# Autodesk Inventor assembly: bike
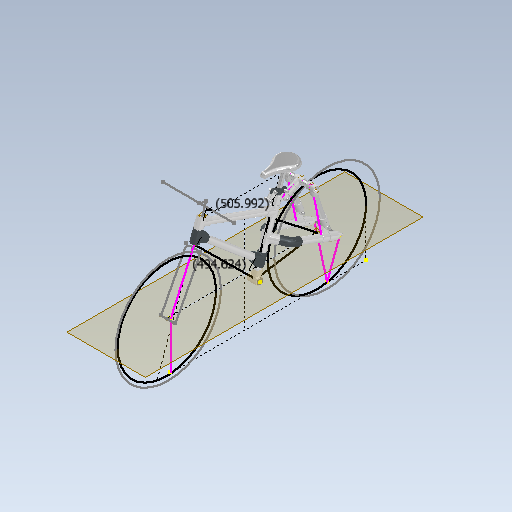
[picture p0: Inventor's stored thumbnail of the model, 512x512]
Saved by Autodesk Inventor 2021 (Build 250183000, 183)
## iProperties
RuleStatus: InUse
Created: 2020-04-29
Part Number: bike
Document SubType Name: Assembly
Designer: Hannah
Mass: 10072.6 g
Surface Area: 13426.9 cm^2
Volume: 2555.77 cm^3
Density: 3.94113 g/cm^3
BeforeDocSave0: estimate cost
Total Cost: 100
Author: Hannah
## Documents named in this file (29)
- \\Mac\Home\Documents\GitHub\AdjustaBike-2.0\CAD\bike.iam
- \\Mac\Home\Documents\GitHub\AdjustaBike-2.0\CAD\prelim bike geo.ipt
- \\Mac\Home\Documents\GitHub\AdjustaBike-2.0\CAD\bottom bracket.ipt
- \\Mac\Home\Documents\GitHub\AdjustaBike-2.0\CAD\L10-7.ipt
- \\Mac\Home\Documents\GitHub\AdjustaBike-2.0\CAD\tube-07.ipt
- \\Mac\Home\Documents\GitHub\AdjustaBike-2.0\CAD\tube-08.ipt
- \\Mac\Home\Documents\GitHub\AdjustaBike-2.0\CAD\tube-11.ipt
- \\Mac\Home\Documents\GitHub\AdjustaBike-2.0\CAD\tube-12.ipt
- \\Mac\Home\Documents\GitHub\AdjustaBike-2.0\CAD\329-7.ipt
- \\Mac\Home\Documents\GitHub\AdjustaBike-2.0\CAD\head tube.ipt
- \\Mac\Home\Documents\GitHub\AdjustaBike-2.0\CAD\LM50-7.ipt
- \\Mac\Home\Documents\GitHub\AdjustaBike-2.0\CAD\LF50-6.ipt
- \\Mac\Home\Documents\GitHub\AdjustaBike-2.0\CAD\55-7.ipt
- \\Mac\Home\Documents\GitHub\AdjustaBike-2.0\CAD\L21-7.ipt
- \\Mac\Home\Documents\GitHub\AdjustaBike-2.0\CAD\tube-13.ipt
- \\Mac\Home\Documents\GitHub\AdjustaBike-2.0\CAD\LF50-7.ipt
- \\Mac\Home\Documents\GitHub\AdjustaBike-2.0\CAD\L10-6.ipt
- \\Mac\Home\Documents\GitHub\AdjustaBike-2.0\CAD\tube-14.ipt
- \\Mac\Home\Documents\GitHub\AdjustaBike-2.0\CAD\L114-6.ipt
- \\Mac\Home\Documents\GitHub\AdjustaBike-2.0\CAD\saddle.ipt
- \\Mac\Home\Documents\GitHub\AdjustaBike-2.0\CAD\M51-5.ipt
- \\Mac\Home\Documents\GitHub\AdjustaBike-2.0\CAD\link.ipt
- \\Mac\Home\Documents\GitHub\AdjustaBike-2.0\CAD\LM51-7.ipt
- \\Mac\Home\Documents\GitHub\AdjustaBike-2.0\CAD\fasteners\DIN 1587 - M10 x 1.5.ipt
- \\Mac\Home\Documents\GitHub\AdjustaBike-2.0\CAD\fasteners\DIN EN ISO 7089 -  10.ipt
- \\Mac\Home\Documents\GitHub\AdjustaBike-2.0\CAD\fasteners\BS EN ISO 4762 - M10 x 35.ipt
- \\Mac\Home\Documents\GitHub\AdjustaBike-2.0\CAD\fasteners\BS EN ISO 4762 - M10 x 45.ipt
- \\Mac\Home\Documents\GitHub\AdjustaBike-2.0\CAD\tube-01.ipt
- \\Mac\Home\Documents\GitHub\AdjustaBike-2.0\CAD\bike sketch.ipt
## Components (69 placed, 28 different names)
1. bike sketch:1 — Flush:126, Flush:127, Flush:128, Mate:236, Mate:237, Mate:238, Mate:239, Mate:240, Mate:241, Mate:242, Mate:243, Mate:244, Mate:245, Mate:246, Mate:247, Mate:248, Mate:249, Mate:250, Mate:251, Mate:252, Mate:253, Mate:254, Mate:255, Mate:256, Mate:257, Mate:258, Mate:259, Mate:260
2. prelim bike geo:1 — Mate:1, Mate:2, Angle:1, Mate:41
3. seat tube:1 — Mate:7, Tangent:1, Flush:9, Angle:2, Mate:8, Angle:5, Mate:17, Tangent:7, Tangent:8, Mate:28, Mate:52, Flush:21, Mate:106, Mate:240
4. down tube:1 — Flush:10, Angle:3, Tangent:2, Mate:11, Tangent:3, Angle:4, Mate:12, Mate:242
5. top tube:1 — Mate:16, Tangent:4, Mate:18, Mate:241
6. seatstay:1 — Mate:91, Mate:93, Mate:97, Mate:245
7. seatstay:2 — Mate:45, Mate:47, Mate:82, Tangent:9, Mate:246
8. seatstay spacer:1 — Mate:89, Mate:90, Mate:92, Mate:100, Tangent:9, Mate:254, Mate:255
9. chainstay:2 — Mate:59, Mate:64, Angle:13, Mate:74, Mate:76, Mate:79, Mate:248
10. chainstay:1 — Mate:58, Mate:62, Angle:12, Mate:75, Mate:77, Mate:247
11. chainstay spacer:1 — Tangent:8, Mate:55, Mate:57, Mate:61, Mate:250
12. chainstay spacer:2 — Tangent:7, Mate:54, Mate:56, Mate:63, Mate:249
13. L10-7:1 — Mate:6, Flush:2, Mate:7, Mate:9
14. L10-7:2 — Mate:17, Mate:18, Mate:261
15. L10-7:3 — Mate:15, Flush:13, Flush:14, Mate:16, Mate:239, Mate:258
16. LM51-7:1 — Mate:28, Flush:16, Mate:69, Flush:20, Flush:21, Flush:22, Mate:107, Mate:110, Mate:111, Mate:112, Mate:113, Mate:114, Mate:204, Mate:261
17. LF50-6:2 — Mate:45, Mate:47, Angle:11, Mate:83, Flush:85, Mate:175
18. L21-7:1 — Mate:52, Mate:53, Mate:54, Mate:55, Mate:60
19. L10-6:3 — Mate:91, Mate:92
20. LF50-6:4 — Mate:93, Mate:95, Mate:96, Mate:97, Mate:150
21. L114-6:1 — Mate:98, Mate:99, Mate:100, Mate:244
22. LF50-6:3 — Mate:69, Flush:20, Mate:98, Mate:99, Mate:108, Mate:109, Mate:232, Mate:243
23. LF50-7:1 — Mate:76, Mate:79, Mate:85, Mate:94, Mate:235, Mate:236, Mate:259
24. LF50-7:2 — Mate:77, Mate:78, Mate:85, Mate:86, Mate:260
25. LM50-7:3 — Mate:75, Mate:83, Flush:85, Mate:86
26. LM50-7:4 — Mate:74, Mate:94, Mate:95, Mate:96
27. L10-6:1 — Mate:82, Mate:89
28. saddle and seatpost:1 — Mate:106, Flush:116
29. head tube:1 — Mate:14, Flush:11, Flush:12, Angle:5, Mate:15, Flush:13, Tangent:4, Mate:237, Mate:257, Mate:262, Mate:263
30. bottom bracket:1 — Mate:4, Flush:1, Mate:5, Mate:6, Tangent:1, Mate:251, Mate:252, Mate:256
31. link:1 — Mate:107, Mate:109, Mate:226, Mate:233
32. link:2 — Mate:111, Mate:113
33. link:3 — Mate:108, Mate:112, Mate:218, Mate:234
34. link:4 — Mate:110, Mate:114, Mate:189
35. DIN 1587 - M10 x 1.5:1 — Mate:162
36. DIN EN ISO 7089 -  10:1
37. BS EN ISO 4762 - M10 x 35:1 — Mate:150, Mate:162
38. DIN EN ISO 7089 -  10:2
39. DIN 1587 - M10 x 1.5:2 — Mate:164
40. DIN EN ISO 7089 -  10:3
41. BS EN ISO 4762 - M10 x 35:2 — Mate:164, Mate:175
42. DIN EN ISO 7089 -  10:4
43. DIN 1587 - M10 x 1.5:3 — Mate:178
44. DIN EN ISO 7089 -  10:5
45. BS EN ISO 4762 - M10 x 35:3 — Mate:178, Mate:189
46. DIN EN ISO 7089 -  10:6
47. DIN 1587 - M10 x 1.5:4 — Mate:201
48. DIN EN ISO 7089 -  10:7
49. BS EN ISO 4762 - M10 x 35:4 — Mate:201, Mate:204
50. DIN EN ISO 7089 -  10:8
51. DIN EN ISO 7089 -  10:11 — Mate:216, Mate:220
52. DIN EN ISO 7089 -  10:12 — Mate:215, Mate:219, Mate:220
53. DIN EN ISO 7089 -  10:13 — Mate:217, Mate:218, Mate:219
54. DIN EN ISO 7089 -  10:14 — Mate:221, Mate:225
55. DIN EN ISO 7089 -  10:15 — Mate:221, Mate:222, Mate:224
56. DIN EN ISO 7089 -  10:16 — Mate:222, Mate:223, Mate:226
57. DIN 1587 - M10 x 1.5:5 — Mate:207
58. DIN EN ISO 7089 -  10:9
59. BS EN ISO 4762 - M10 x 45:1 — Mate:207, Mate:212, Mate:215, Mate:216, Mate:217, Mate:223, Mate:224, Mate:225
60. DIN EN ISO 7089 -  10:10
61. DIN 1587 - M10 x 1.5:6 — Mate:227, Mate:230
62. DIN EN ISO 7089 -  10:17 — Mate:228, Mate:229, Mate:234
63. BS EN ISO 4762 - M10 x 45:2 — Mate:227, Mate:228, Mate:229, Mate:231, Mate:232
64. DIN EN ISO 7089 -  10:18 — Mate:230, Mate:231, Mate:233, Mate:253
65. 329-7:1 — Mate:8, Mate:9, Mate:10, Angle:3, Tangent:2, Mate:11, Mate:53
66. 329-7:2 — Tangent:3, Angle:4, Mate:12, Mate:13, Mate:14, Flush:11, Mate:238
67. 55-7:1 — Mate:56, Mate:59, Mate:63, Mate:64
68. 55-7:2 — Mate:57, Mate:58, Mate:61, Mate:62
69. M51-5:1 — Mate:212
## Relationships (196: Mate 163, Flush 18, Angle 8, Tangent 7)
- Mate:1: prelim bike geo:1
- Mate:2: prelim bike geo:1
- Mate:3
- Mate:4: bottom bracket:1
- Flush:1: bottom bracket:1
- Angle:1 (0 deg): prelim bike geo:1
- Mate:5: bottom bracket:1
- Mate:6: L10-7:1 ↔ bottom bracket:1
- Flush:2: L10-7:1
- Mate:7: seat tube:1 ↔ L10-7:1
- Tangent:1: seat tube:1 ↔ bottom bracket:1
- Flush:9: seat tube:1
- Angle:2 (-70 deg): seat tube:1
- Flush:10: down tube:1
- Mate:8: seat tube:1 ↔ 329-7:1
- Mate:9 (5 mm): L10-7:1 ↔ 329-7:1
- Mate:10: 329-7:1
- Angle:3 (72 deg): down tube:1 ↔ 329-7:1
- Tangent:2: down tube:1 ↔ 329-7:1
- Mate:11: down tube:1 ↔ 329-7:1
- Tangent:3: down tube:1 ↔ 329-7:2
- Angle:4 (0 deg): down tube:1 ↔ 329-7:2
- Mate:12: down tube:1 ↔ 329-7:2
- Mate:13: 329-7:2
- Mate:14: head tube:1 ↔ 329-7:2
- Flush:11: head tube:1 ↔ 329-7:2
- Flush:12: head tube:1
- Angle:5 (0 deg): seat tube:1 ↔ head tube:1
- Mate:15: L10-7:3 ↔ head tube:1
- Flush:13: L10-7:3 ↔ head tube:1
- Flush:14: L10-7:3
- Mate:16: top tube:1 ↔ L10-7:3
- Tangent:4: top tube:1 ↔ head tube:1
- Mate:17: seat tube:1 ↔ L10-7:2
- Mate:18: top tube:1 ↔ L10-7:2
- Tangent:7: seat tube:1 ↔ chainstay spacer:2
- Tangent:8: seat tube:1 ↔ chainstay spacer:1
- Mate:28: seat tube:1 ↔ LM51-7:1
- Flush:16: LM51-7:1
- Mate:41: prelim bike geo:1
- Mate:45: seatstay:2 ↔ LF50-6:2
- Mate:47: seatstay:2 ↔ LF50-6:2
- Angle:11 (0 deg): LF50-6:2
- Mate:52: seat tube:1 ↔ L21-7:1
- Mate:53 (5 mm): L21-7:1 ↔ 329-7:1
- Mate:54: chainstay spacer:2 ↔ L21-7:1
- Mate:55: chainstay spacer:1 ↔ L21-7:1
- Mate:56: chainstay spacer:2 ↔ 55-7:1
- Mate:57: chainstay spacer:1 ↔ 55-7:2
- Mate:58: chainstay:1 ↔ 55-7:2
- Mate:59: chainstay:2 ↔ 55-7:1
- Mate:60: L21-7:1
- Mate:61 (-35 mm): chainstay spacer:1 ↔ 55-7:2
- Mate:62 (-35 mm): chainstay:1 ↔ 55-7:2
- Mate:63 (-35 mm): chainstay spacer:2 ↔ 55-7:1
- Mate:64 (-35 mm): chainstay:2 ↔ 55-7:1
- Angle:12 (0 deg): chainstay:1
- Angle:13 (0 deg): chainstay:2
- Mate:69: LM51-7:1 ↔ LF50-6:3
- Flush:20: LM51-7:1 ↔ LF50-6:3
- Flush:21: seat tube:1 ↔ LM51-7:1
- Mate:74: chainstay:2 ↔ LM50-7:4
- Mate:75: chainstay:1 ↔ LM50-7:3
- Mate:76: chainstay:2 ↔ LF50-7:1
- Mate:77: chainstay:1 ↔ LF50-7:2
- Mate:78: LF50-7:2
- Mate:79: chainstay:2 ↔ LF50-7:1
- Flush:22: LM51-7:1
- Mate:82: seatstay:2 ↔ L10-6:1
- Mate:83: LF50-6:2 ↔ LM50-7:3
- Flush:85: LF50-6:2 ↔ LM50-7:3
- Mate:85: LF50-7:1 ↔ LF50-7:2
- Mate:86 (5 mm): LF50-7:2 ↔ LM50-7:3
- Mate:89: seatstay spacer:1 ↔ L10-6:1
- Mate:90: seatstay spacer:1
- Mate:91: seatstay:1 ↔ L10-6:3
- Mate:92: seatstay spacer:1 ↔ L10-6:3
- Mate:93: seatstay:1 ↔ LF50-6:4
- Mate:94 (5 mm): LF50-7:1 ↔ LM50-7:4
- Mate:95: LF50-6:4 ↔ LM50-7:4
- Mate:96: LF50-6:4 ↔ LM50-7:4
- Mate:97: seatstay:1 ↔ LF50-6:4
- Mate:98: L114-6:1 ↔ LF50-6:3
- Mate:99: L114-6:1 ↔ LF50-6:3
- Mate:100: seatstay spacer:1 ↔ L114-6:1
- Tangent:9: seatstay:2 ↔ seatstay spacer:1
- [Mate]: saddle and seatpost:1 ↔ M51-5:1
- [Mate]: link:3 ↔ M51-5:1
- [Mate]: link:4 ↔ M51-5:1
- [Mate]: link:2 ↔ M51-5:1
- [Mate]: link:1 ↔ M51-5:1
- Mate:106: seat tube:1 ↔ saddle and seatpost:1
- Mate:107: LM51-7:1 ↔ link:1
- Mate:108: LF50-6:3 ↔ link:3
- Mate:109: LF50-6:3 ↔ link:1
- Mate:110: LM51-7:1 ↔ link:4
- Mate:111: LM51-7:1 ↔ link:2
- Mate:112: LM51-7:1 ↔ link:3
- Mate:113: LM51-7:1 ↔ link:2
- Mate:114: LM51-7:1 ↔ link:4
- Flush:116: saddle and seatpost:1
- Mate:150: LF50-6:4 ↔ BS EN ISO 4762 - M10 x 35:1
- [Mate]: DIN EN ISO 7089 -  10:1 ↔ BS EN ISO 4762 - M10 x 35:1
- [Mate]: DIN EN ISO 7089 -  10:1 ↔ BS EN ISO 4762 - M10 x 35:1
- [Mate]: LF50-6:4 ↔ DIN EN ISO 7089 -  10:1
- [Mate]: BS EN ISO 4762 - M10 x 35:1 ↔ DIN EN ISO 7089 -  10:2
- [Mate]: LF50-6:4 ↔ DIN EN ISO 7089 -  10:2
- Mate:162: DIN 1587 - M10 x 1.5:1 ↔ BS EN ISO 4762 - M10 x 35:1
- Mate:164: DIN 1587 - M10 x 1.5:2 ↔ BS EN ISO 4762 - M10 x 35:2
- [Mate]: DIN EN ISO 7089 -  10:3 ↔ BS EN ISO 4762 - M10 x 35:2
- [Mate]: DIN EN ISO 7089 -  10:3 ↔ BS EN ISO 4762 - M10 x 35:2
- [Mate]: BS EN ISO 4762 - M10 x 35:2 ↔ DIN EN ISO 7089 -  10:4
- Mate:175: LF50-6:2 ↔ BS EN ISO 4762 - M10 x 35:2
- [Mate]: LF50-6:2 ↔ DIN EN ISO 7089 -  10:3
- [Mate]: LF50-6:2 ↔ DIN EN ISO 7089 -  10:4
- Mate:178: DIN 1587 - M10 x 1.5:3 ↔ BS EN ISO 4762 - M10 x 35:3
- [Mate]: DIN EN ISO 7089 -  10:5 ↔ BS EN ISO 4762 - M10 x 35:3
- [Mate]: DIN EN ISO 7089 -  10:5 ↔ BS EN ISO 4762 - M10 x 35:3
- [Mate]: BS EN ISO 4762 - M10 x 35:3 ↔ DIN EN ISO 7089 -  10:6
- Mate:189: link:4 ↔ BS EN ISO 4762 - M10 x 35:3
- [Mate]: link:4 ↔ DIN EN ISO 7089 -  10:5
- [Mate]: link:2 ↔ DIN EN ISO 7089 -  10:6
- [Mate]: DIN 1587 - M10 x 1.5:1 ↔ DIN EN ISO 7089 -  10:2
- [Mate]: DIN 1587 - M10 x 1.5:2 ↔ DIN EN ISO 7089 -  10:4
- [Mate]: DIN 1587 - M10 x 1.5:3 ↔ DIN EN ISO 7089 -  10:6
- [Mate]: DIN EN ISO 7089 -  10:7 ↔ BS EN ISO 4762 - M10 x 35:4
- [Mate]: DIN EN ISO 7089 -  10:7 ↔ BS EN ISO 4762 - M10 x 35:4
- Mate:201: DIN 1587 - M10 x 1.5:4 ↔ BS EN ISO 4762 - M10 x 35:4
- [Mate]: DIN 1587 - M10 x 1.5:4 ↔ DIN EN ISO 7089 -  10:8
- [Mate]: BS EN ISO 4762 - M10 x 35:4 ↔ DIN EN ISO 7089 -  10:8
- Mate:204: LM51-7:1 ↔ BS EN ISO 4762 - M10 x 35:4
- [Mate]: link:4 ↔ DIN EN ISO 7089 -  10:7
- [Mate]: link:2 ↔ DIN EN ISO 7089 -  10:8
- Mate:207: DIN 1587 - M10 x 1.5:5 ↔ BS EN ISO 4762 - M10 x 45:1
- [Mate]: DIN EN ISO 7089 -  10:9 ↔ BS EN ISO 4762 - M10 x 45:1
- [Mate]: DIN EN ISO 7089 -  10:9 ↔ BS EN ISO 4762 - M10 x 45:1
- [Mate]: BS EN ISO 4762 - M10 x 45:1 ↔ DIN EN ISO 7089 -  10:10
- [Mate]: DIN 1587 - M10 x 1.5:5 ↔ DIN EN ISO 7089 -  10:10
- Mate:212: BS EN ISO 4762 - M10 x 45:1 ↔ M51-5:1
- [Mate]: link:3 ↔ DIN EN ISO 7089 -  10:9
- [Mate]: link:1 ↔ DIN EN ISO 7089 -  10:10
- Mate:215: DIN EN ISO 7089 -  10:12 ↔ BS EN ISO 4762 - M10 x 45:1
- Mate:216: DIN EN ISO 7089 -  10:11 ↔ BS EN ISO 4762 - M10 x 45:1
- Mate:217: DIN EN ISO 7089 -  10:13 ↔ BS EN ISO 4762 - M10 x 45:1
- Mate:218: link:3 ↔ DIN EN ISO 7089 -  10:13
- Mate:219: DIN EN ISO 7089 -  10:12 ↔ DIN EN ISO 7089 -  10:13
- Mate:220: DIN EN ISO 7089 -  10:11 ↔ DIN EN ISO 7089 -  10:12
- Mate:221: DIN EN ISO 7089 -  10:14 ↔ DIN EN ISO 7089 -  10:15
- Mate:222: DIN EN ISO 7089 -  10:15 ↔ DIN EN ISO 7089 -  10:16
- Mate:223: DIN EN ISO 7089 -  10:16 ↔ BS EN ISO 4762 - M10 x 45:1
- Mate:224: DIN EN ISO 7089 -  10:15 ↔ BS EN ISO 4762 - M10 x 45:1
- Mate:225: DIN EN ISO 7089 -  10:14 ↔ BS EN ISO 4762 - M10 x 45:1
- Mate:226: link:1 ↔ DIN EN ISO 7089 -  10:16
- Mate:227: DIN 1587 - M10 x 1.5:6 ↔ BS EN ISO 4762 - M10 x 45:2
- Mate:228: DIN EN ISO 7089 -  10:17 ↔ BS EN ISO 4762 - M10 x 45:2
- Mate:229: DIN EN ISO 7089 -  10:17 ↔ BS EN ISO 4762 - M10 x 45:2
- Mate:230: DIN 1587 - M10 x 1.5:6 ↔ DIN EN ISO 7089 -  10:18
- Mate:231: BS EN ISO 4762 - M10 x 45:2 ↔ DIN EN ISO 7089 -  10:18
- Mate:232: LF50-6:3 ↔ BS EN ISO 4762 - M10 x 45:2
- Mate:233: link:1 ↔ DIN EN ISO 7089 -  10:18
- Mate:234: link:3 ↔ DIN EN ISO 7089 -  10:17
- Flush:126: bike sketch:1
- Flush:127: bike sketch:1
- Flush:128: bike sketch:1
- Flush:129 (60 mm)
- Mate:235: LF50-7:1
- Mate:236: bike sketch:1 ↔ LF50-7:1
- Mate:237: bike sketch:1 ↔ head tube:1
- Mate:238: bike sketch:1 ↔ 329-7:2
- Mate:239: bike sketch:1 ↔ L10-7:3
- Mate:240: bike sketch:1 ↔ seat tube:1
- Mate:241: bike sketch:1 ↔ top tube:1
- Mate:242: bike sketch:1 ↔ down tube:1
- Mate:243: bike sketch:1 ↔ LF50-6:3
- Mate:244: bike sketch:1 ↔ L114-6:1
- Mate:245: bike sketch:1 ↔ seatstay:1
- Mate:246: bike sketch:1 ↔ seatstay:2
- Mate:247: bike sketch:1 ↔ chainstay:1
- Mate:248: bike sketch:1 ↔ chainstay:2
- Mate:249: bike sketch:1 ↔ chainstay spacer:2
- Mate:250: bike sketch:1 ↔ chainstay spacer:1
- Mate:251: bike sketch:1 ↔ bottom bracket:1
- Mate:252: bike sketch:1 ↔ bottom bracket:1
- Mate:253: bike sketch:1 ↔ DIN EN ISO 7089 -  10:18
- Mate:254: bike sketch:1 ↔ seatstay spacer:1
- Mate:255: bike sketch:1 ↔ seatstay spacer:1
- Mate:256: bike sketch:1 ↔ bottom bracket:1
- Mate:257: bike sketch:1 ↔ head tube:1
- Mate:258: bike sketch:1 ↔ L10-7:3
- Mate:259: bike sketch:1 ↔ LF50-7:1
- Mate:260: bike sketch:1 ↔ LF50-7:2
- Mate:261 (5 mm): L10-7:2 ↔ LM51-7:1
- Mate:262: head tube:1
- Mate:263: head tube:1
- Mate:264 (568 mm)
- Mate:265 (376 mm)
## Named parameters: Lst = 440 mm, Sst = 7, Ldt = 494 mm, Sdt = 7, Ltt = 505 mm, Stt = 7, Lcs = 300 mm, Scs = 7, Lss = 234 mm, Sss = 6, Lsp = 80 mm, Ssp = 7, Scsn = 7, Lspn = 234 mm, d166_d164 = 0 mm, stack = 568 mm, reach = 376 mm, BBdrop = 60 mm, TTLength = 505.99187 mm, DTLength = 494.62414 mm
